# Autodesk Inventor assembly: magnet_assembly_rear
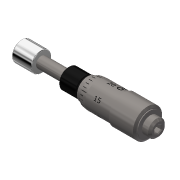
[picture p0: Inventor's stored thumbnail of the model, 180x180]
Saved by Autodesk Inventor 2019 (Build 230136000, 136)
## iProperties
Created: 2023-10-12
Part Number: magnet_assembly_rear
Document SubType Name: Assembly
Designer: prich
Author: prich
## Documents named in this file (3)
- C:\Users\prich\Dropbox\Princeton\Project\head_fixation\cad_models\magnet_assembly_rear.iam
- C:\Users\prich\Dropbox\Princeton\Project\head_fixation\cad_models\148-202FT-H-Step.ipt
- C:\Users\prich\Dropbox\Princeton\Project\head_fixation\cad_models\D44-N52.ipt
## Components (2 placed, 2 different names)
1. 148-202FT-H-Step:1 — Insert:1
2. D44-N52:1 — Insert:1
## Relationships (1: Insert 1)
- Insert:1: 148-202FT-H-Step:1 ↔ D44-N52:1
